# Autodesk Inventor assembly: FullUnitAssembly
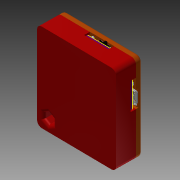
[picture p0: Inventor's stored thumbnail of the model, 180x180]
Saved by Autodesk Inventor 2015 SP2 (Build 190223200, 223)
## iProperties
Created: 2016-07-22
Part Number: FullUnitAssembly
Document SubType Name: Assembly
Designer: Iain
Author: Iain
## Documents named in this file (5)
- D:\Sit-To-Stand\BLEVibrator\Hardware\Case\FullUnitAssembly.iam
- D:\Sit-To-Stand\BLEVibrator\Hardware\Case\CaseBottom.ipt
- D:\Sit-To-Stand\BLEVibrator\Hardware\Case\CaseTop.ipt
- D:\Sit-To-Stand\BLEVibrator\Hardware\Case\308-106.ipt
- D:\Sit-To-Stand\BLEVibrator\Hardware\Case\PCBAssembly.iam
## Components (4 placed, 4 different names)
1. CaseBottom:1 — Flush:4, Mate:2, Flush:1, Symmetry:1, Insert:1, Mate:3, Flush:2, Flush:3
2. CaseTop:1 — Flush:4, Mate:2, Flush:1, Symmetry:1
3. 308-106:1 — Insert:1
4. PCBAssembly:1 [sub-assembly] — Mate:3, Flush:2, Flush:3
## Relationships (8: Flush 4, Mate 2, Symmetry 1, Insert 1)
- Flush:4: CaseBottom:1 ↔ CaseTop:1
- Mate:2: CaseBottom:1 ↔ CaseTop:1
- Flush:1: CaseBottom:1 ↔ CaseTop:1
- Symmetry:1: CaseBottom:1 ↔ CaseTop:1
- Insert:1 (0.1 mm): CaseBottom:1 ↔ 308-106:1
- Mate:3: CaseBottom:1 ↔ PCBAssembly:1
- Flush:2 (0.5 mm): CaseBottom:1 ↔ PCBAssembly:1
- Flush:3 (0.5 mm): CaseBottom:1 ↔ PCBAssembly:1
